# Autodesk Inventor assembly: detectionObjAssembly
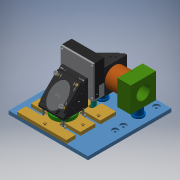
[picture p0: Inventor's stored thumbnail of the model, 180x180]
Saved by Autodesk Inventor 2016 (Build 200138000, 138)
## iProperties
Created: 2016-03-08
Part Number: detectionObjAssembly
Document SubType Name: Assembly
Designer: sims01
Author: sims01
## Documents named in this file (15)
- H:\Documents\LSFM_3\setup\mechanical\design\lsfm3_mechDesign\detectionObjAssembly.iam
- H:\Documents\LSFM_3\setup\mechanical\design\lsfm3_mechDesign\detectionObjHolder.ipt
- H:\Documents\LSFM_3\setup\mechanical\design\lsfm3_mechDesign\cageRodHolder.ipt
- H:\Documents\LSFM_3\setup\mechanical\design\lsfm3_mechDesign\25mmCageRod.ipt
- H:\Documents\LSFM_3\setup\mechanical\design\lsfm3_mechDesign\rectangularObjectiveHolder.ipt
- H:\Documents\LSFM_3\setup\mechanical\design\lsfm3_mechDesign\cylindricalObjectiveHolder.ipt
- H:\Documents\LSFM_3\setup\mechanical\design\lsfm3_mechDesign\olympusXLSLPLN25XGMP_vFIN.ipt
- H:\Documents\LSFM_3\setup\mechanical\design\lsfm3_mechDesign\45degEllipticalMirrorAssembly.iam
- H:\Documents\LSFM_3\setup\mechanical\design\lsfm3_mechDesign\25mmPedestalPost.ipt
- H:\Documents\LSFM_3\setup\mechanical\design\lsfm3_mechDesign\1mmPostSpacer.ipt
- H:\Documents\LSFM_3\setup\mechanical\design\lsfm3_mechDesign\0.7mmPostSpacer.ipt
- H:\Documents\LSFM_3\setup\mechanical\design\lsfm3_mechDesign\cairnFilterWheel.iam
- H:\Documents\LSFM_3\setup\mechanical\design\lsfm3_mechDesign\44.8mmOpticalPost.ipt
- H:\Documents\LSFM_3\setup\mechanical\design\lsfm3_mechDesign\tubeLensHolder.ipt
- H:\Documents\LSFM_3\setup\mechanical\design\lsfm3_mechDesign\olympusTubeLens.ipt
## Components (25 placed, 14 different names)
1. detectionObjHolder:1 — Rigid:1, Rigid:2, Rigid:3, Rigid:4, Rigid:10, Rigid:16, Rotational:22, Rotational:23
2. cageRodHolder:1 — Rigid:2, Rigid:12
3. cageRodHolder:2 — Rigid:3, Rigid:14
4. cageRodHolder:3 — Rigid:4, Rigid:15
5. cageRodHolder:4 — Rigid:1, Rigid:13
6. 25mmCageRod:1 — Rigid:14
7. 25mmCageRod:2 — Rigid:13
8. 25mmCageRod:3 — Rigid:12, Rotational:1
9. 25mmCageRod:4 — Rigid:15
10. rectangularObjectiveHolder:1 — Rigid:9, Rigid:10
11. cylindricalObjectiveHolder:1 — Rigid:9, Rigid:11
12. olympusXLSLPLN25XGMP_vFIN:1 — Rigid:11
13. 45degEllipticalMirrorAssembly:1 [sub-assembly] — Rotational:1
14. 25mmPedestalPost:1 — Rigid:16, Rigid:17
15. 1mmPostSpacer:1 — Rigid:17, Rigid:18
16. 0.7mmPostSpacer:1 — Rigid:18, Rotational:2
17. 45degEllipticalMirrorAssembly:2 [sub-assembly] — Rotational:2
18. cairnFilterWheel:1 [sub-assembly] — Rigid:19, Rigid:20
19. 44.8mmOpticalPost:1 — Rigid:20
20. 44.8mmOpticalPost:2 — Rigid:19, Rotational:22
21. tubeLensHolder:1 — Rigid:21, Rigid:24
22. olympusTubeLens:1 — Rigid:21
23. 25mmPedestalPost:2 — Rotational:23
24. 1mmPostSpacer:2
25. 0.7mmPostSpacer:2 — Rigid:24
## Relationships (24: WeldJoint 20, RevoluteJoint 4)
- Rigid:1 [WeldJoint]: detectionObjHolder:1 ↔ cageRodHolder:4
- Rigid:2 [WeldJoint]: detectionObjHolder:1 ↔ cageRodHolder:1
- Rigid:3 [WeldJoint]: detectionObjHolder:1 ↔ cageRodHolder:2
- Rigid:4 [WeldJoint]: detectionObjHolder:1 ↔ cageRodHolder:3
- Rigid:9 [WeldJoint]: rectangularObjectiveHolder:1 ↔ cylindricalObjectiveHolder:1
- Rigid:10 [WeldJoint]: detectionObjHolder:1 ↔ rectangularObjectiveHolder:1
- Rigid:11 [WeldJoint]: cylindricalObjectiveHolder:1 ↔ olympusXLSLPLN25XGMP_vFIN:1
- Rigid:12 [WeldJoint]: cageRodHolder:1 ↔ 25mmCageRod:3
- Rigid:13 [WeldJoint]: cageRodHolder:4 ↔ 25mmCageRod:2
- Rigid:14 [WeldJoint]: cageRodHolder:2 ↔ 25mmCageRod:1
- Rigid:15 [WeldJoint]: cageRodHolder:3 ↔ 25mmCageRod:4
- Rotational:1 [RevoluteJoint]: 25mmCageRod:3 ↔ 45degEllipticalMirrorAssembly:1
- Rigid:16 [WeldJoint]: detectionObjHolder:1 ↔ 25mmPedestalPost:1
- Rigid:17 [WeldJoint]: 25mmPedestalPost:1 ↔ 1mmPostSpacer:1
- Rigid:18 [WeldJoint]: 1mmPostSpacer:1 ↔ 0.7mmPostSpacer:1
- Rotational:2 [RevoluteJoint]: 0.7mmPostSpacer:1 ↔ 45degEllipticalMirrorAssembly:2
- Rigid:19 [WeldJoint]: cairnFilterWheel:1 ↔ 44.8mmOpticalPost:2
- Rigid:20 [WeldJoint]: cairnFilterWheel:1 ↔ 44.8mmOpticalPost:1
- Rotational:22 [RevoluteJoint]: detectionObjHolder:1 ↔ 44.8mmOpticalPost:2
- Rigid:21 [WeldJoint]: tubeLensHolder:1 ↔ olympusTubeLens:1
- [WeldJoint]: 25mmPedestalPost:2 ↔ 1mmPostSpacer:2
- [WeldJoint]: 1mmPostSpacer:2 ↔ 0.7mmPostSpacer:2
- Rigid:24 [WeldJoint]: tubeLensHolder:1 ↔ 0.7mmPostSpacer:2
- Rotational:23 [RevoluteJoint]: detectionObjHolder:1 ↔ 25mmPedestalPost:2
## Named parameters: d68_d27 = 0 mm, d69_d28 = 0 mm
